# Autodesk Inventor assembly: アームアセンブリ2
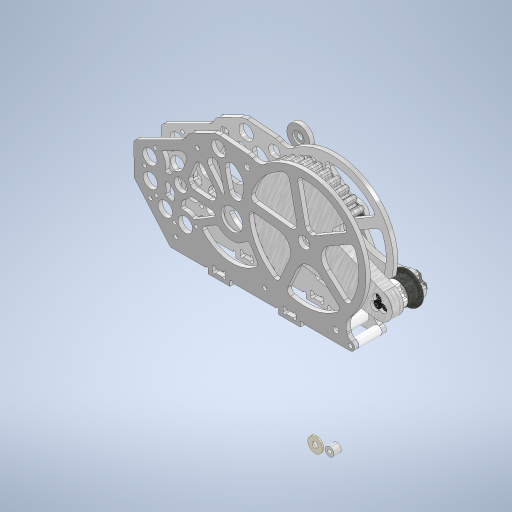
[picture p0: Inventor's stored thumbnail of the model, 512x512]
Saved by Autodesk Inventor 2023 (Build 270158030, 158C)
## iProperties
Created: 2022-06-19
Part Number: アームアセンブリ2
Document SubType Name: Assembly
Designer: muzho
Author: muzho
## Documents named in this file (16)
- C:\Users\muzho\Documents\srdc\srdc_2\アーム\アームアセンブリ2.iam
- C:\Users\muzho\Documents\srdc\srdc_2\アーム\主フレーム.ipt
- C:\Users\muzho\Documents\srdc\srdc_2\アーム\右フレーム.ipt
- C:\Users\muzho\Documents\srdc\srdc_2\アーム(世古)\既製品\スペーサーm4-35　簡易筒型.ipt
- C:\Users\muzho\Documents\srdc\srdc_2\アーム(世古)\既製品\スペーサーm3-16　簡易筒型.ipt
- C:\Users\muzho\Documents\srdc\srdc_2\アーム\左フレーム.ipt
- C:\Users\muzho\Documents\srdc\srdc_2\アーム\ギア\最終段m2z40.ipt
- C:\Users\muzho\Documents\srdc\srdc_2\アーム(世古)\アーム 駆動フリー節.ipt
- C:\Users\muzho\Documents\srdc\srdc_2\スペーサ\l5.ipt
- C:\Users\muzho\Documents\srdc\srdc_2\ワッシャー\チタンワッシャー　4.2-10-1.ipt
- C:\Users\muzho\Documents\srdc\srdc_2\オイレス\w3f6-8a.ipt
- C:\Users\muzho\Documents\srdc\srdc_2\アーム(世古)\アーム 小さいカム押さえるやつ.ipt
- C:\Users\muzho\Documents\srdc\srdc_2\ねじ\M3ボタンボルト25.ipt
- C:\Users\muzho\Documents\srdc\srdc_2\アーム(世古)\アーム 小さいカム.ipt
- C:\Users\muzho\Documents\srdc\srdc_2\アーム(世古)\既製品\ドライメット　内径14 フランジ付き6mm.ipt
- C:\Users\muzho\Documents\srdc\srdc_2\ねじ\ナイロンナットm3.ipt
## Components (19 placed, 15 different names)
1. 主フレーム:1 — メイト:1, メイト:2, 挿入:3, メイト:3, メイト:4
2. 右フレーム:1 — メイト:1, メイト:2, 挿入:1, 挿入:2, メイト:5
3. スペーサーm3-16　簡易筒型:1 — 挿入:1, 挿入:3
4. スペーサーm4-35　簡易筒型:1 — 挿入:2, 挿入:4
5. 左フレーム:1 — メイト:3, メイト:4, 挿入:4, メイト:6, 挿入:5
6. 最終段m2z40:1 — メイト:5, メイト:7, メイト:8, メイト:9, 挿入:6, 挿入:7, 挿入:8, 挿入:9
7. アーム 駆動フリー節:1 — メイト:6, メイト:7, 挿入:12, 挿入:13, 挿入:14, 挿入:15
8. l5:1
9. チタンワッシャー　4.2-10-1:1
10. w3f6-8a:1 — 挿入:5
11. アーム 小さいカム押さえるやつ:1 — メイト:8, メイト:9, 挿入:6, 挿入:10
12. M3ボタンボルト25:1 — 挿入:7, メイト:10
13. M3ボタンボルト25:2 — 挿入:8, メイト:11
14. M3ボタンボルト25:3 — 挿入:9
15. アーム 小さいカム:1 — メイト:10, メイト:11, 挿入:10, 挿入:11, 挿入:12
16. ドライメット　内径14 フランジ付き6mm:1 — 挿入:11
17. ナイロンナットm3:1 — 挿入:14, メイト:12, メイト:13
18. ナイロンナットm3:2 — 挿入:15, メイト:13
19. ナイロンナットm3:3 — 挿入:13, メイト:12
## Relationships (28: Insert 15, Mate 13)
- メイト:1 [Mate]: 主フレーム:1 ↔ 右フレーム:1
- メイト:2 [Mate]: 主フレーム:1 ↔ 右フレーム:1
- 挿入:1 [Insert]: 右フレーム:1 ↔ スペーサーm3-16　簡易筒型:1
- 挿入:2 [Insert]: 右フレーム:1 ↔ スペーサーm4-35　簡易筒型:1
- 挿入:3 [Insert]: 主フレーム:1 ↔ スペーサーm3-16　簡易筒型:1
- メイト:3 [Mate]: 主フレーム:1 ↔ 左フレーム:1
- メイト:4 [Mate]: 主フレーム:1 ↔ 左フレーム:1
- 挿入:4 [Insert]: スペーサーm4-35　簡易筒型:1 ↔ 左フレーム:1
- メイト:5 [Mate]: 右フレーム:1 ↔ 最終段m2z40:1
- メイト:6 [Mate]: 左フレーム:1 ↔ アーム 駆動フリー節:1
- 挿入:5 [Insert]: 左フレーム:1 ↔ w3f6-8a:1
- メイト:7 [Mate]: 最終段m2z40:1 ↔ アーム 駆動フリー節:1
- メイト:8 [Mate]: 最終段m2z40:1 ↔ アーム 小さいカム押さえるやつ:1
- メイト:9 [Mate]: 最終段m2z40:1 ↔ アーム 小さいカム押さえるやつ:1
- 挿入:6 [Insert]: 最終段m2z40:1 ↔ アーム 小さいカム押さえるやつ:1
- 挿入:7 [Insert]: 最終段m2z40:1 ↔ M3ボタンボルト25:1
- 挿入:8 [Insert]: 最終段m2z40:1 ↔ M3ボタンボルト25:2
- 挿入:9 [Insert]: 最終段m2z40:1 ↔ M3ボタンボルト25:3
- メイト:10 [Mate]: M3ボタンボルト25:1 ↔ アーム 小さいカム:1
- メイト:11 [Mate]: M3ボタンボルト25:2 ↔ アーム 小さいカム:1
- 挿入:10 [Insert]: アーム 小さいカム押さえるやつ:1 ↔ アーム 小さいカム:1
- 挿入:11 [Insert] (0.5 mm): アーム 小さいカム:1 ↔ ドライメット　内径14 フランジ付き6mm:1
- 挿入:12 [Insert]: アーム 駆動フリー節:1 ↔ アーム 小さいカム:1
- 挿入:13 [Insert]: アーム 駆動フリー節:1 ↔ ナイロンナットm3:3
- 挿入:14 [Insert]: アーム 駆動フリー節:1 ↔ ナイロンナットm3:1
- 挿入:15 [Insert]: アーム 駆動フリー節:1 ↔ ナイロンナットm3:2
- メイト:12 [Mate]: ナイロンナットm3:1 ↔ ナイロンナットm3:3
- メイト:13 [Mate]: ナイロンナットm3:1 ↔ ナイロンナットm3:2
